# Autodesk Inventor assembly: elevator
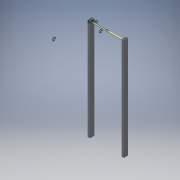
[picture p0: Inventor's stored thumbnail of the model, 180x180]
Saved by Autodesk Inventor 2017 (Build 210142000, 142)
## iProperties
Created: 2017-12-27
Part Number: elevator
Document SubType Name: Assembly
Designer: Micah
Author: Micah
## Documents named in this file (6)
- C:\Users\Micah\Desktop\inventor\CADathon-2017\Assemblies\2AM-17-A-0200.iam
- C:\Users\Micah\Desktop\inventor\CADathon-2017\Parts\2AM-17-A-0200 - Smokestack Elevator\2AM-17-P-0201.ipt
- C:\Users\Micah\Desktop\inventor\CADathon-2017\COTS\0_500_Hex_ID_x_1_125_OD_x_0_313_WD_Flanged_Bearing_v2_217-3875.ipt
- C:\Users\Micah\Desktop\inventor\CADathon-2017\Parts\2AM-17-A-0200 - Smokestack Elevator\2AM-17-P-0204.ipt
- C:\Users\Micah\Desktop\inventor\CADathon-2017\COTS\217-2737.20121205.ipt
- C:\Users\Micah\Desktop\inventor\CADathon-2017\COTS\_22t_Aluminum_Hub_Sprocket_25_Chain_1_2_Hex_Bore_217-2640.ipt
## Components (9 placed, 5 different names)
1. 2AM-17-P-0201:2 — Mate:4
2. 2AM-17-P-0201:3 — Mate:5
3. 0_500_Hex_ID_x_1_125_OD_x_0_313_WD_Flanged_Bearing_v2_217-3875:1 — Mate:4, Rigid:1
4. 0_500_Hex_ID_x_1_125_OD_x_0_313_WD_Flanged_Bearing_v2_217-3875:2 — Mate:5
5. 2AM-17-P-0204:1 — Rigid:1, Rigid:2, Rigid:3, Mate:6
6. 217-2737.20121205:1 — Rigid:2
7. 217-2737.20121205:2 — Rigid:3
8. _22t_Aluminum_Hub_Sprocket_25_Chain_1_2_Hex_Bore_217-2640:1 — Mate:6
9. _22t_Aluminum_Hub_Sprocket_25_Chain_1_2_Hex_Bore_217-2640:2
## Relationships (6: Mate 3, WeldJoint 3)
- Mate:4: 2AM-17-P-0201:2 ↔ 0_500_Hex_ID_x_1_125_OD_x_0_313_WD_Flanged_Bearing_v2_217-3875:1
- Mate:5: 2AM-17-P-0201:3 ↔ 0_500_Hex_ID_x_1_125_OD_x_0_313_WD_Flanged_Bearing_v2_217-3875:2
- Rigid:1 [WeldJoint] (-14.2875 mm): 0_500_Hex_ID_x_1_125_OD_x_0_313_WD_Flanged_Bearing_v2_217-3875:1 ↔ 2AM-17-P-0204:1
- Rigid:2 [WeldJoint]: 2AM-17-P-0204:1 ↔ 217-2737.20121205:1
- Rigid:3 [WeldJoint]: 2AM-17-P-0204:1 ↔ 217-2737.20121205:2
- Mate:6: 2AM-17-P-0204:1 ↔ _22t_Aluminum_Hub_Sprocket_25_Chain_1_2_Hex_Bore_217-2640:1
